# Autodesk Inventor assembly: wheelsys
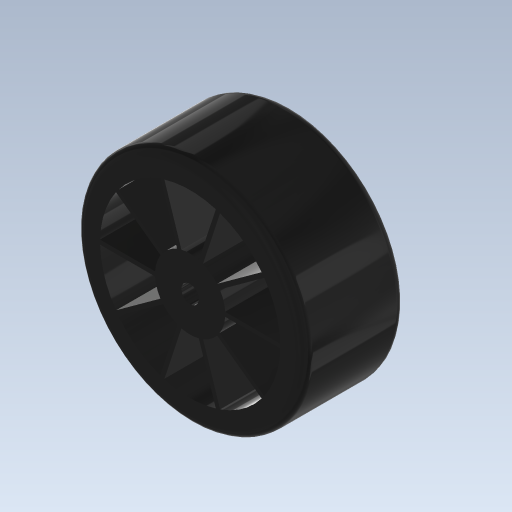
[picture p0: Inventor's stored thumbnail of the model, 512x512]
Saved by Autodesk Inventor 2023 (Build 270158000, 158)
## iProperties
Created: 2023-05-04
Part Number: wheelsys
Document SubType Name: Assembly
Designer: Johnny Jou
Author: Johnny Jou
## Documents named in this file (5)
- C:\Users\Johnny Jou\Documents\GitHub\Areo_Rider_Cabin\car\wheelsys.iam
- C:\Users\Johnny Jou\Documents\GitHub\Areo_Rider_Cabin\car\wheel.ipt
- C:\Users\Johnny Jou\Documents\GitHub\Areo_Rider_Cabin\car\Coupling_0515.ipt
- C:\Users\Johnny Jou\Documents\GitHub\Areo_Rider_Cabin\car\2GT_40T.ipt
- C:\Users\Johnny Jou\Documents\GitHub\Areo_Rider_Cabin\car\2GTbase.ipt
## Components (4 placed, 4 different names)
1. wheel:1 — 貼合:13, 貼合:14
2. Coupling_0515:1 — 貼合:13, 貼合:14, 貼合:15, 貼合:16, 貼合:17, 貼合:18, 貼合:19
3. 2GT_40T:1 — 貼合:15, 貼合:16, 貼合:17, 貼合:20
4. 2GTbase:1 — 貼合:18, 貼合:19, 貼合:20
## Relationships (8: Mate 8)
- 貼合:13 [Mate]: wheel:1 ↔ Coupling_0515:1
- 貼合:14 [Mate]: wheel:1 ↔ Coupling_0515:1
- 貼合:15 [Mate]: Coupling_0515:1 ↔ 2GT_40T:1
- 貼合:16 [Mate]: Coupling_0515:1 ↔ 2GT_40T:1
- 貼合:17 [Mate]: Coupling_0515:1 ↔ 2GT_40T:1
- 貼合:18 [Mate]: Coupling_0515:1 ↔ 2GTbase:1
- 貼合:19 [Mate]: Coupling_0515:1 ↔ 2GTbase:1
- 貼合:20 [Mate]: 2GT_40T:1 ↔ 2GTbase:1
